# Autodesk Inventor assembly: ArcadeController
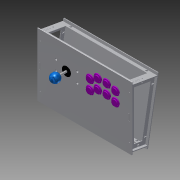
[picture p0: Inventor's stored thumbnail of the model, 180x180]
Saved by Autodesk Inventor 2013 (Build 170138000, 138)
## iProperties
Created: 2013-02-02
Part Number: ArcadeController
Document SubType Name: Assembly
Designer: xylzlyx
Author: xylzlyx
## Documents named in this file (13)
- C:\dev\pewpew\assemblies\ArcadeController.iam
- C:\dev\pewpew\parts\Panel_top.ipt
- C:\dev\pewpew\parts\Panel_bottom.ipt
- C:\dev\pewpew\parts\JLF-TP-8YT_body.ipt
- C:\dev\pewpew\parts\JLF-TP-8YT_ball.ipt
- C:\dev\pewpew\parts\JLF-TP-8YT_ring.ipt
- C:\dev\pewpew\parts\OBSF-30-B_button.ipt
- C:\dev\pewpew\assemblies\ArcadeController\Design Accelerator\Bolted Connection1.iam
- C:\dev\pewpew\parts\Panel_back.ipt
- C:\dev\pewpew\parts\Panel_front.ipt
- C:\dev\pewpew\parts\Panel_side.ipt
- C:\Users\xylzlyx\Documents\Inventor\Content Center Files\R2013\en-US\ANSI B18.3(05)\ANSI B18.3 - 6-32 UNC - 0.5(31).ipt
- C:\Users\xylzlyx\Documents\Inventor\Content Center Files\R2013\en-US\ANSI B18.22.1\ANSI B18.22.1 - No. 6 - Type A.ipt
## Components (50 placed, 12 different names)
1. TopPanel:1 — Flush:1, Flush:2, Insert:1, Insert:2, Insert:4, Insert:5, Insert:6, Insert:7, Insert:8, Insert:9, Insert:10, Insert:11, Insert:12, Mate:1, Mate:2, Mate:6, Mate:10, Insert:14, Insert:17, Insert:18, Insert:19
2. BottomPanel:1 — Flush:1, Flush:2, Mate:3, Flush:3, Flush:4, Flush:5, Flush:6, Flush:8, Flush:9, Mate:4, Mate:5, Flush:10, Flush:12, Flush:13, Mate:8, Flush:14, Mate:13, Insert:22, Insert:23, Insert:24, Insert:25, Insert:26, Insert:27, Insert:28, Insert:29
3. JLF-TP-8YT_body:1 — Insert:1, Insert:2, Insert:3, Mate:3
4. JoystickBall:1 — Insert:3
5. JoystickCover:1 — Insert:4
6. OBSF-30-B_button:1 — Insert:5
7. OBSF-30-B_button:2 — Insert:6
8. OBSF-30-B_button:3 — Insert:7
9. OBSF-30-B_button:4 — Insert:8
10. OBSF-30-B_button:5 — Insert:9
11. OBSF-30-B_button:6 — Insert:10
12. OBSF-30-B_button:7 — Insert:11
13. OBSF-30-B_button:8 — Insert:12
14. Bolted Connection:1 [sub-assembly] — Mate:1, Mate:2
15. Panel_back:1 — Flush:3, Flush:4, Mate:5, Flush:10, Mate:11, Mate:12, Insert:15, Insert:16
16. Panel_front:1 — Flush:5, Flush:6, Flush:12, Mate:9, Flush:14, Mate:13, Insert:20, Insert:21
17. Panel_side:1 — Flush:8, Flush:9, Mate:4, Mate:6, Mate:12
18. Panel_side:2 — Flush:13, Mate:8, Mate:9, Mate:10, Mate:11
19. Hexagon Socket Head Cap Screw - Inch No. 6 - 32 UNC - 1/2:4 — Insert:13
20. Plain Washer (Inch) No. 6 - Type A:1 — Insert:13, Insert:14
21. Hexagon Socket Head Cap Screw - Inch No. 6 - 32 UNC - 1/2:5 — Insert:30
22. Plain Washer (Inch) No. 6 - Type A:2 — Insert:15, Insert:31
23. Hexagon Socket Head Cap Screw - Inch No. 6 - 32 UNC - 1/2:6 — Insert:31
24. Plain Washer (Inch) No. 6 - Type A:3 — Insert:16, Insert:30
25. Hexagon Socket Head Cap Screw - Inch No. 6 - 32 UNC - 1/2:7 — Insert:32
26. Plain Washer (Inch) No. 6 - Type A:4 — Insert:17, Insert:35
27. Hexagon Socket Head Cap Screw - Inch No. 6 - 32 UNC - 1/2:8 — Insert:33
28. Plain Washer (Inch) No. 6 - Type A:5 — Insert:19, Insert:32
29. Hexagon Socket Head Cap Screw - Inch No. 6 - 32 UNC - 1/2:9 — Insert:34
30. Plain Washer (Inch) No. 6 - Type A:6 — Insert:18, Insert:34
31. Plain Washer (Inch) No. 6 - Type A:7 — Insert:20, Insert:33
32. Plain Washer (Inch) No. 6 - Type A:8 — Insert:21, Insert:36
33. Plain Washer (Inch) No. 6 - Type A:9 — Insert:25, Insert:43
34. Plain Washer (Inch) No. 6 - Type A:10 — Insert:24, Insert:44
35. Plain Washer (Inch) No. 6 - Type A:11 — Insert:23, Insert:39
36. Plain Washer (Inch) No. 6 - Type A:12 — Insert:22, Insert:40
37. Plain Washer (Inch) No. 6 - Type A:13 — Insert:26, Insert:37
38. Plain Washer (Inch) No. 6 - Type A:14 — Insert:27, Insert:38
39. Plain Washer (Inch) No. 6 - Type A:15 — Insert:28, Insert:41
40. Plain Washer (Inch) No. 6 - Type A:16 — Insert:29, Insert:42
41. Hexagon Socket Head Cap Screw - Inch No. 6 - 32 UNC - 1/2:10 — Insert:40
42. Hexagon Socket Head Cap Screw - Inch No. 6 - 32 UNC - 1/2:11 — Insert:35
43. Hexagon Socket Head Cap Screw - Inch No. 6 - 32 UNC - 1/2:12 — Insert:36
44. Hexagon Socket Head Cap Screw - Inch No. 6 - 32 UNC - 1/2:13 — Insert:37
45. Hexagon Socket Head Cap Screw - Inch No. 6 - 32 UNC - 1/2:14 — Insert:39
46. Hexagon Socket Head Cap Screw - Inch No. 6 - 32 UNC - 1/2:15 — Insert:38
47. Hexagon Socket Head Cap Screw - Inch No. 6 - 32 UNC - 1/2:16 — Insert:42
48. Hexagon Socket Head Cap Screw - Inch No. 6 - 32 UNC - 1/2:17 — Insert:41
49. Hexagon Socket Head Cap Screw - Inch No. 6 - 32 UNC - 1/2:18 — Insert:43
50. Hexagon Socket Head Cap Screw - Inch No. 6 - 32 UNC - 1/2:19 — Insert:44
## Relationships (68: Insert 44, Flush 12, Mate 12)
- Flush:1: TopPanel:1 ↔ BottomPanel:1
- Flush:2: TopPanel:1 ↔ BottomPanel:1
- Insert:1: TopPanel:1 ↔ JLF-TP-8YT_body:1
- Insert:2: TopPanel:1 ↔ JLF-TP-8YT_body:1
- Insert:3: JLF-TP-8YT_body:1 ↔ JoystickBall:1
- Insert:4: TopPanel:1 ↔ JoystickCover:1
- Insert:5: TopPanel:1 ↔ OBSF-30-B_button:1
- Insert:6: TopPanel:1 ↔ OBSF-30-B_button:2
- Insert:7: TopPanel:1 ↔ OBSF-30-B_button:3
- Insert:8: TopPanel:1 ↔ OBSF-30-B_button:4
- Insert:9: TopPanel:1 ↔ OBSF-30-B_button:5
- Insert:10: TopPanel:1 ↔ OBSF-30-B_button:6
- Insert:11: TopPanel:1 ↔ OBSF-30-B_button:7
- Insert:12: TopPanel:1 ↔ OBSF-30-B_button:8
- Mate:1: TopPanel:1 ↔ Bolted Connection:1
- Mate:2: TopPanel:1 ↔ Bolted Connection:1
- Mate:3 (44.45 mm): BottomPanel:1 ↔ JLF-TP-8YT_body:1
- Flush:3: BottomPanel:1 ↔ Panel_back:1
- Flush:4 (-12.7 mm): BottomPanel:1 ↔ Panel_back:1
- Flush:5: BottomPanel:1 ↔ Panel_front:1
- Flush:6 (-9.525 mm): BottomPanel:1 ↔ Panel_front:1
- Flush:8 (-9.525 mm): BottomPanel:1 ↔ Panel_side:1
- Flush:9 (9.525 mm): BottomPanel:1 ↔ Panel_side:1
- Mate:4: BottomPanel:1 ↔ Panel_side:1
- Mate:5: BottomPanel:1 ↔ Panel_back:1
- Flush:10: BottomPanel:1 ↔ Panel_back:1
- Mate:6: TopPanel:1 ↔ Panel_side:1
- Flush:12 (9.525 mm): BottomPanel:1 ↔ Panel_front:1
- Flush:13 (9.525 mm): BottomPanel:1 ↔ Panel_side:2
- Mate:8: BottomPanel:1 ↔ Panel_side:2
- Mate:9: Panel_front:1 ↔ Panel_side:2
- Mate:10: TopPanel:1 ↔ Panel_side:2
- Mate:11: Panel_back:1 ↔ Panel_side:2
- Mate:12: Panel_back:1 ↔ Panel_side:1
- Flush:14: BottomPanel:1 ↔ Panel_front:1
- Mate:13: BottomPanel:1 ↔ Panel_front:1
- Insert:13: Hexagon Socket Head Cap Screw - Inch No. 6 - 32 UNC - 1/2:4 ↔ Plain Washer (Inch) No. 6 - Type A:1
- Insert:14: TopPanel:1 ↔ Plain Washer (Inch) No. 6 - Type A:1
- Insert:15: Panel_back:1 ↔ Plain Washer (Inch) No. 6 - Type A:2
- Insert:16: Panel_back:1 ↔ Plain Washer (Inch) No. 6 - Type A:3
- Insert:17: TopPanel:1 ↔ Plain Washer (Inch) No. 6 - Type A:4
- Insert:18: TopPanel:1 ↔ Plain Washer (Inch) No. 6 - Type A:6
- Insert:19: TopPanel:1 ↔ Plain Washer (Inch) No. 6 - Type A:5
- Insert:20: Panel_front:1 ↔ Plain Washer (Inch) No. 6 - Type A:7
- Insert:21: Panel_front:1 ↔ Plain Washer (Inch) No. 6 - Type A:8
- Insert:22: BottomPanel:1 ↔ Plain Washer (Inch) No. 6 - Type A:12
- Insert:23: BottomPanel:1 ↔ Plain Washer (Inch) No. 6 - Type A:11
- Insert:24: BottomPanel:1 ↔ Plain Washer (Inch) No. 6 - Type A:10
- Insert:25: BottomPanel:1 ↔ Plain Washer (Inch) No. 6 - Type A:9
- Insert:26: BottomPanel:1 ↔ Plain Washer (Inch) No. 6 - Type A:13
- Insert:27: BottomPanel:1 ↔ Plain Washer (Inch) No. 6 - Type A:14
- Insert:28: BottomPanel:1 ↔ Plain Washer (Inch) No. 6 - Type A:15
- Insert:29: BottomPanel:1 ↔ Plain Washer (Inch) No. 6 - Type A:16
- Insert:30: Hexagon Socket Head Cap Screw - Inch No. 6 - 32 UNC - 1/2:5 ↔ Plain Washer (Inch) No. 6 - Type A:3
- Insert:31: Plain Washer (Inch) No. 6 - Type A:2 ↔ Hexagon Socket Head Cap Screw - Inch No. 6 - 32 UNC - 1/2:6
- Insert:32: Hexagon Socket Head Cap Screw - Inch No. 6 - 32 UNC - 1/2:7 ↔ Plain Washer (Inch) No. 6 - Type A:5
- Insert:33: Hexagon Socket Head Cap Screw - Inch No. 6 - 32 UNC - 1/2:8 ↔ Plain Washer (Inch) No. 6 - Type A:7
- Insert:34: Hexagon Socket Head Cap Screw - Inch No. 6 - 32 UNC - 1/2:9 ↔ Plain Washer (Inch) No. 6 - Type A:6
- Insert:35: Plain Washer (Inch) No. 6 - Type A:4 ↔ Hexagon Socket Head Cap Screw - Inch No. 6 - 32 UNC - 1/2:11
- Insert:36: Plain Washer (Inch) No. 6 - Type A:8 ↔ Hexagon Socket Head Cap Screw - Inch No. 6 - 32 UNC - 1/2:12
- Insert:37: Plain Washer (Inch) No. 6 - Type A:13 ↔ Hexagon Socket Head Cap Screw - Inch No. 6 - 32 UNC - 1/2:13
- Insert:38: Plain Washer (Inch) No. 6 - Type A:14 ↔ Hexagon Socket Head Cap Screw - Inch No. 6 - 32 UNC - 1/2:15
- Insert:39: Plain Washer (Inch) No. 6 - Type A:11 ↔ Hexagon Socket Head Cap Screw - Inch No. 6 - 32 UNC - 1/2:14
- Insert:40: Plain Washer (Inch) No. 6 - Type A:12 ↔ Hexagon Socket Head Cap Screw - Inch No. 6 - 32 UNC - 1/2:10
- Insert:41: Plain Washer (Inch) No. 6 - Type A:15 ↔ Hexagon Socket Head Cap Screw - Inch No. 6 - 32 UNC - 1/2:17
- Insert:42: Plain Washer (Inch) No. 6 - Type A:16 ↔ Hexagon Socket Head Cap Screw - Inch No. 6 - 32 UNC - 1/2:16
- Insert:43: Plain Washer (Inch) No. 6 - Type A:9 ↔ Hexagon Socket Head Cap Screw - Inch No. 6 - 32 UNC - 1/2:18
- Insert:44: Plain Washer (Inch) No. 6 - Type A:10 ↔ Hexagon Socket Head Cap Screw - Inch No. 6 - 32 UNC - 1/2:19
